# Autodesk Inventor assembly: ASSEMBLY
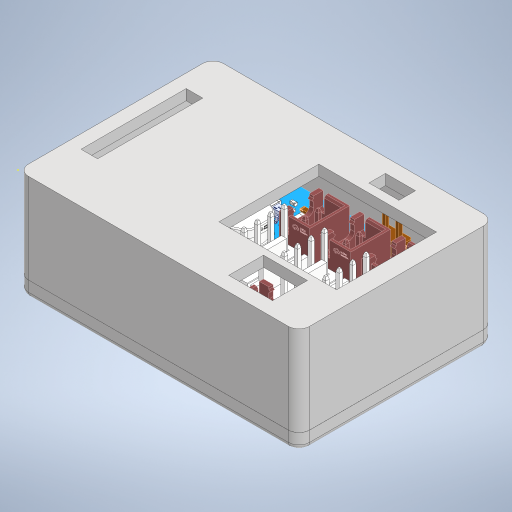
[picture p0: Inventor's stored thumbnail of the model, 512x512]
Saved by Autodesk Inventor 2023 (Build 270158000, 158)
## iProperties
Created: 2023-10-08
Part Number: ASSEMBLY
Document SubType Name: Assembly
Designer: a laptop
Author: a laptop
## Documents named in this file (4)
- C:\Users\a laptop\Desktop\Stm8_Fancontroller\CAD\ASSEMBLY.iam
- C:\Users\a laptop\Desktop\Stm8_Fancontroller\CAD\Frame_Bottom.ipt
- C:\Users\a laptop\Desktop\Stm8_Fancontroller\CAD\3D_PCB_fancontroller_Fullpartdetail_2023-10-08.iam
- C:\Users\a laptop\Desktop\Stm8_Fancontroller\CAD\Frame_Lid.ipt
## Components (3 placed, 3 different names)
1. Frame_Bottom:1 — Mate:1, Angle:1, Mate:2, Flush:1, Flush:2, Mate:3
2. 3D_PCB_fancontroller_Fullpartdetail_2023-10-08:1 [sub-assembly] — Mate:1, Angle:1, Mate:2
3. Frame_Lid:1 — Flush:1, Flush:2, Mate:3
## Relationships (6: Mate 3, Flush 2, Angle 1)
- Mate:1: Frame_Bottom:1 ↔ 3D_PCB_fancontroller_Fullpartdetail_2023-10-08:1
- Angle:1 (0 deg): Frame_Bottom:1 ↔ 3D_PCB_fancontroller_Fullpartdetail_2023-10-08:1
- Mate:2 (2 mm): Frame_Bottom:1 ↔ 3D_PCB_fancontroller_Fullpartdetail_2023-10-08:1
- Flush:1: Frame_Bottom:1 ↔ Frame_Lid:1
- Flush:2: Frame_Bottom:1 ↔ Frame_Lid:1
- Mate:3: Frame_Bottom:1 ↔ Frame_Lid:1
